# Autodesk Inventor assembly: hopper_assy
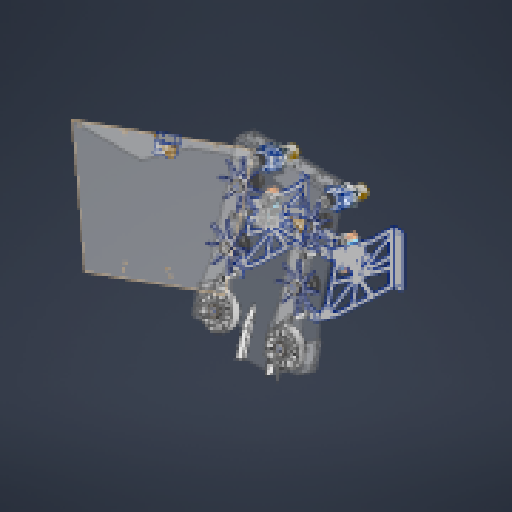
[picture p0: Inventor's stored thumbnail of the model, 512x512]
Saved by Autodesk Inventor 2024.3 (Build 283343000, 343)
## iProperties
Created: 2025-03-15
Part Number: hopper_assy
Document SubType Name: Assembly
Designer: Marcus Tannini
Author: Marcus Tannini
## Documents named in this file (31)
- C:\Users\jings\OneDrive\Desktop\FRC 5885\2025-Poseidon-Mechanical\hopper_assy.iam
- C:\Users\jings\OneDrive\Desktop\FRC 5885\2025-Poseidon-Mechanical\hopper_side_l.ipt
- C:\Users\jings\OneDrive\Desktop\FRC 5885\2025-Poseidon-Mechanical\hopper_side_r.ipt
- C:\Users\jings\OneDrive\Desktop\FRC 5885\2025-Poseidon-Mechanical\feeder_bottom_plate.ipt
- C:\Users\jings\OneDrive\Desktop\FRC 5885\2025-Poseidon-Mechanical\hopper_back.ipt
- C:\Users\jings\OneDrive\Desktop\FRC 5885\2025-Poseidon-Mechanical\hopper_side_bracket.ipt
- C:\Users\jings\OneDrive\Desktop\FRC 5885\2025-Poseidon-Mechanical\feeder_guide_plate.ipt
- C:\Users\jings\OneDrive\Desktop\FRC 5885\2025-Poseidon-Mechanical\am-5123 5IN 500IN Hex Bore Compliant Star.iam
- C:\Users\jings\OneDrive\Desktop\FRC 5885\2025-Poseidon-Mechanical\feeder_guide_plate_MIR.ipt
- C:\Users\jings\OneDrive\Desktop\FRC 5885\2025-Poseidon-Mechanical\CONTROLS,MOTOR,NEO,550.ipt
- C:\Users\jings\OneDrive\Desktop\FRC 5885\2025-Poseidon-Mechanical\VersaPlanetary v2 Dual Stage 10_1 with RS 550 (1).iam
- C:\Users\jings\OneDrive\Desktop\FRC 5885\2025-Poseidon-Mechanical\coral_guide.ipt
- C:\Users\jings\OneDrive\Desktop\FRC 5885\2025-Poseidon-Mechanical\coral_guide_MIR.ipt
- C:\Users\jings\OneDrive\Desktop\FRC 5885\2025-Poseidon-Mechanical\feeder_side_support_r.ipt
- C:\Users\jings\OneDrive\Desktop\FRC 5885\2025-Poseidon-Mechanical\feeder_side_support_l.ipt
- C:\Users\jings\OneDrive\Desktop\FRC 5885\2025-Poseidon-Mechanical\feeder_middle_brace.ipt
- C:\Users\jings\OneDrive\Desktop\FRC 5885\2025-Poseidon-Mechanical\2_1-2_hex_shaft.ipt
- C:\Users\jings\OneDrive\Desktop\FRC 5885\2025-Poseidon-Mechanical\PURCHASED,HEX_BEARING.ipt
- C:\Users\jings\OneDrive\Desktop\FRC 5885\2025-Poseidon-Mechanical\Bolt_Spacer.ipt
- C:\Users\jings\OneDrive\Desktop\FRC 5885\2025-Poseidon-Mechanical\CONTROLS,SPARK_MAX.ipt
- C:\Users\jings\OneDrive\Desktop\FRC 5885\2025-Poseidon-Mechanical\COVER,SPARKMAX.ipt
- C:\Users\jings\OneDrive\Desktop\FRC 5885\2025-Poseidon-Mechanical\16t 9mm.ipt
- C:\Users\jings\OneDrive\Desktop\FRC 5885\2025-Poseidon-Mechanical\19t 9mm.ipt
- C:\Users\jings\OneDrive\Desktop\FRC 5885\2025-Poseidon-Mechanical\29t 9mm.ipt
- C:\Users\jings\OneDrive\Desktop\FRC 5885\2025-Poseidon-Mechanical\am-3480 4IN 500Hex Bore Compliant Wheel REV2(1).iam
- C:\Users\jings\OneDrive\Desktop\FRC 5885\2025-Poseidon-Mechanical\1-2in_spacer.ipt
- C:\Users\jings\OneDrive\Desktop\FRC 5885\2025-Poseidon-Mechanical\hopper_fin.ipt
- C:\Users\jings\OneDrive\Desktop\FRC 5885\2025-Poseidon-Mechanical\hopper_fin_MIR.ipt
- C:\Users\jings\OneDrive\Desktop\FRC 5885\2025-Poseidon-Mechanical\1_CAD Library\CONTROLS,SPARK_MAX.ipt
- C:\Users\jings\OneDrive\Desktop\FRC 5885\2025-Poseidon-Mechanical\1_CAD Library\PURCHASED,GEARBOX,VERSA_PLANETARY,ADAPTER_CIM.ipt
- C:\Users\jings\OneDrive\Desktop\FRC 5885\2025-Poseidon-Mechanical\1_CAD Library\CONTROLS,MOTOR,NEO,V1.ipt
## Components (73 placed, 29 different names)
1. hopper_side_l:1
2. hopper_side_r:1
3. feeder_bottom_plate:1 — Mate:170, Mate:171, Mate:172, Mate:173, Mate:174, Mate:175
4. hopper_back:1
5. hopper_side_bracket:1
6. hopper_side_bracket:2
7. feeder_guide_plate:1
8. am-5123 5IN 500IN Hex Bore Compliant Star:1 [sub-assembly]
9. feeder_guide_plate_MIR:1
10. CONTROLS,MOTOR,NEO,550:1
11. VersaPlanetary v2 Dual Stage 10_1 with RS 550 (1):1 [sub-assembly]
12. coral_guide:1
13. coral_guide_MIR:1
14. feeder_side_support_r:1 — Mate:170, Mate:171, Mate:172
15. feeder_side_support_l:1 — Mate:173, Mate:174, Mate:175
16. feeder_middle_brace:1
17. 2_1-2_hex_shaft:1
18. PURCHASED,HEX_BEARING:1
19. 2_1-2_hex_shaft:2
20. PURCHASED,HEX_BEARING:2
21. am-5123 5IN 500IN Hex Bore Compliant Star:2 [sub-assembly]
22. 2_1-2_hex_shaft:3
23. PURCHASED,HEX_BEARING:3
24. am-5123 5IN 500IN Hex Bore Compliant Star:3 [sub-assembly]
25. 2_1-2_hex_shaft:4
26. PURCHASED,HEX_BEARING:4
27. am-5123 5IN 500IN Hex Bore Compliant Star:4 [sub-assembly]
28. CONTROLS,MOTOR,NEO,550:2
29. VersaPlanetary v2 Dual Stage 10_1 with RS 550 (1):2 [sub-assembly]
30. PURCHASED,HEX_BEARING:5
31. PURCHASED,HEX_BEARING:6
32. PURCHASED,HEX_BEARING:7
33. PURCHASED,HEX_BEARING:8
34. Bolt_Spacer:1
35. Bolt_Spacer:2
36. CONTROLS,SPARK_MAX:1
37. COVER,SPARKMAX:1
38. CONTROLS,SPARK_MAX:2
39. COVER,SPARKMAX:2
40. PURCHASED,HEX_BEARING:9
41. 2_1-2_hex_shaft:5
42. 2_1-2_hex_shaft:6
43. PURCHASED,HEX_BEARING:10
44. PURCHASED,HEX_BEARING:11
45. PURCHASED,HEX_BEARING:12
46. 16t 9mm:1
47. 16t 9mm:2
48. 16t 9mm:3
49. 16t 9mm:4
50. 19t 9mm:1
51. 19t 9mm:2
52. 19t 9mm:3
53. 19t 9mm:4
54. 29t 9mm:1
55. 29t 9mm:2
56. 29t 9mm:3
57. 29t 9mm:4
58. Bolt_Spacer:3
59. Bolt_Spacer:4
60. am-3480 4IN 500Hex Bore Compliant Wheel REV2(1):1 [sub-assembly]
61. am-3480 4IN 500Hex Bore Compliant Wheel REV2(1):2 [sub-assembly]
62. 1-2in_spacer:1
63. 1-2in_spacer:2
64. 1-2in_spacer:3
65. 1-2in_spacer:4
66. 1-2in_spacer:5
67. 1-2in_spacer:6
68. hopper_fin:1
69. hopper_fin_MIR:1
70. CONTROLS,SPARK_MAX:3
71. PURCHASED,GEARBOX,VERSA_PLANETARY,ADAPTER_CIM:1 — Insert:1, Insert:2, Insert:3, Insert:4
72. CONTROLS,MOTOR,NEO,V1:1 — Insert:1, Insert:2
73. VersaPlanetary v2 Dual Stage 10_1 with RS 550 (1):3 [sub-assembly] — Insert:3, Insert:4
## Relationships (197: Mate 168, Flush 20, RelateRotation 5, Insert 4)
- [Mate]: feeder_bottom_plate:1 ↔ hopper_back:1
- [Mate]: feeder_bottom_plate:1 ↔ hopper_back:1
- [Mate]: feeder_bottom_plate:1 ↔ hopper_back:1
- [Mate]: hopper_back:1 ↔ hopper_side_bracket:1
- [Mate]: hopper_back:1 ↔ hopper_side_bracket:1
- [Mate]: hopper_back:1 ↔ hopper_side_bracket:1
- [Mate]: hopper_side_l:1 ↔ hopper_side_bracket:1
- [Mate]: hopper_side_l:1 ↔ hopper_side_bracket:1
- [Mate]: hopper_side_l:1 ↔ hopper_side_bracket:1
- [Mate]: hopper_back:1 ↔ hopper_side_bracket:2
- [Mate]: hopper_back:1 ↔ hopper_side_bracket:2
- [Mate]: hopper_back:1 ↔ hopper_side_bracket:2
- [Mate]: hopper_side_r:1 ↔ hopper_side_bracket:2
- [Mate]: hopper_side_r:1 ↔ hopper_side_bracket:2
- [Mate]: hopper_side_r:1 ↔ hopper_side_bracket:2
- [Mate]: feeder_bottom_plate:1 ↔ feeder_guide_plate:1
- [Mate]: feeder_bottom_plate:1 ↔ feeder_guide_plate_MIR:1
- [Mate]: CONTROLS,MOTOR,NEO,550:1 ↔ VersaPlanetary v2 Dual Stage 10_1 with RS 550 (1):1
- [Mate]: CONTROLS,MOTOR,NEO,550:1 ↔ VersaPlanetary v2 Dual Stage 10_1 with RS 550 (1):1
- [Mate]: feeder_bottom_plate:1 ↔ VersaPlanetary v2 Dual Stage 10_1 with RS 550 (1):1
- [Flush]: feeder_bottom_plate:1 ↔ coral_guide:1
- [Mate]: feeder_bottom_plate:1 ↔ coral_guide:1
- [Flush]: feeder_bottom_plate:1 ↔ coral_guide_MIR:1
- [Mate]: feeder_bottom_plate:1 ↔ coral_guide_MIR:1
- [Mate] (69.85 mm): coral_guide:1 ↔ coral_guide_MIR:1
- [Flush] (11.1125 mm): feeder_bottom_plate:1 ↔ coral_guide:1
- [Mate]: feeder_side_support_r:1 ↔ feeder_middle_brace:1
- [Mate]: feeder_side_support_r:1 ↔ feeder_middle_brace:1
- [Mate]: feeder_side_support_r:1 ↔ feeder_middle_brace:1
- [Mate]: 2_1-2_hex_shaft:1 ↔ PURCHASED,HEX_BEARING:1
- [Mate]: 2_1-2_hex_shaft:1 ↔ PURCHASED,HEX_BEARING:1
- [Flush]: 2_1-2_hex_shaft:1 ↔ PURCHASED,HEX_BEARING:1
- [Mate]: 2_1-2_hex_shaft:2 ↔ PURCHASED,HEX_BEARING:2
- [Mate]: 2_1-2_hex_shaft:2 ↔ PURCHASED,HEX_BEARING:2
- [Flush]: 2_1-2_hex_shaft:2 ↔ PURCHASED,HEX_BEARING:2
- [Mate]: 2_1-2_hex_shaft:1 ↔ am-5123 5IN 500IN Hex Bore Compliant Star:2
- [Mate]: 2_1-2_hex_shaft:1 ↔ am-5123 5IN 500IN Hex Bore Compliant Star:2
- [Mate]: PURCHASED,HEX_BEARING:1 ↔ am-5123 5IN 500IN Hex Bore Compliant Star:2
- [Mate]: feeder_bottom_plate:1 ↔ feeder_guide_plate:1
- [Mate]: feeder_bottom_plate:1 ↔ feeder_guide_plate_MIR:1
- [Mate]: 2_1-2_hex_shaft:3 ↔ PURCHASED,HEX_BEARING:3
- [Mate]: 2_1-2_hex_shaft:3 ↔ PURCHASED,HEX_BEARING:3
- [Flush]: 2_1-2_hex_shaft:3 ↔ PURCHASED,HEX_BEARING:3
- [Mate]: 2_1-2_hex_shaft:3 ↔ am-5123 5IN 500IN Hex Bore Compliant Star:3
- [Mate]: 2_1-2_hex_shaft:3 ↔ am-5123 5IN 500IN Hex Bore Compliant Star:3
- [Mate]: PURCHASED,HEX_BEARING:3 ↔ am-5123 5IN 500IN Hex Bore Compliant Star:3
- [Mate]: 2_1-2_hex_shaft:4 ↔ PURCHASED,HEX_BEARING:4
- [Mate]: 2_1-2_hex_shaft:4 ↔ PURCHASED,HEX_BEARING:4
- [Flush]: 2_1-2_hex_shaft:4 ↔ PURCHASED,HEX_BEARING:4
- [Mate]: CONTROLS,MOTOR,NEO,550:2 ↔ VersaPlanetary v2 Dual Stage 10_1 with RS 550 (1):2
- [Mate]: CONTROLS,MOTOR,NEO,550:2 ↔ VersaPlanetary v2 Dual Stage 10_1 with RS 550 (1):2
- [Mate]: feeder_bottom_plate:1 ↔ VersaPlanetary v2 Dual Stage 10_1 with RS 550 (1):2
- [Mate]: feeder_bottom_plate:1 ↔ Bolt_Spacer:1
- [Mate]: feeder_bottom_plate:1 ↔ Bolt_Spacer:1
- [Mate]: feeder_bottom_plate:1 ↔ Bolt_Spacer:2
- [Mate]: feeder_bottom_plate:1 ↔ Bolt_Spacer:2
- [Mate]: CONTROLS,SPARK_MAX:1 ↔ COVER,SPARKMAX:1
- [Mate]: CONTROLS,SPARK_MAX:1 ↔ COVER,SPARKMAX:1
- [Mate]: CONTROLS,SPARK_MAX:1 ↔ COVER,SPARKMAX:1
- [Mate]: CONTROLS,SPARK_MAX:2 ↔ COVER,SPARKMAX:2
- [Mate]: CONTROLS,SPARK_MAX:2 ↔ COVER,SPARKMAX:2
- [Mate]: CONTROLS,SPARK_MAX:2 ↔ COVER,SPARKMAX:2
- [Mate]: feeder_side_support_r:1 ↔ COVER,SPARKMAX:1
- [Mate]: feeder_side_support_r:1 ↔ COVER,SPARKMAX:1
- [Mate]: feeder_side_support_r:1 ↔ CONTROLS,SPARK_MAX:1
- [Mate]: feeder_side_support_l:1 ↔ COVER,SPARKMAX:2
- [Mate]: feeder_side_support_l:1 ↔ COVER,SPARKMAX:2
- [Mate]: feeder_side_support_l:1 ↔ CONTROLS,SPARK_MAX:2
- [Mate]: feeder_bottom_plate:1 ↔ VersaPlanetary v2 Dual Stage 10_1 with RS 550 (1):1
- [Mate]: feeder_bottom_plate:1 ↔ VersaPlanetary v2 Dual Stage 10_1 with RS 550 (1):1
- [Mate]: feeder_bottom_plate:1 ↔ VersaPlanetary v2 Dual Stage 10_1 with RS 550 (1):2
- [Mate]: feeder_bottom_plate:1 ↔ VersaPlanetary v2 Dual Stage 10_1 with RS 550 (1):2
- [Mate]: PURCHASED,HEX_BEARING:9 ↔ 2_1-2_hex_shaft:6
- [Mate]: PURCHASED,HEX_BEARING:9 ↔ 2_1-2_hex_shaft:6
- [Flush]: PURCHASED,HEX_BEARING:9 ↔ 2_1-2_hex_shaft:6
- [Flush]: 2_1-2_hex_shaft:6 ↔ PURCHASED,HEX_BEARING:12
- [Mate]: 2_1-2_hex_shaft:6 ↔ PURCHASED,HEX_BEARING:12
- [Mate]: 2_1-2_hex_shaft:6 ↔ PURCHASED,HEX_BEARING:12
- [Flush]: 2_1-2_hex_shaft:5 ↔ PURCHASED,HEX_BEARING:10
- [Mate]: 2_1-2_hex_shaft:5 ↔ PURCHASED,HEX_BEARING:10
- [Mate]: 2_1-2_hex_shaft:5 ↔ PURCHASED,HEX_BEARING:10
- [Flush]: 2_1-2_hex_shaft:5 ↔ PURCHASED,HEX_BEARING:11
- [Mate]: 2_1-2_hex_shaft:5 ↔ PURCHASED,HEX_BEARING:11
- [Mate]: 2_1-2_hex_shaft:5 ↔ PURCHASED,HEX_BEARING:11
- [Mate]: feeder_guide_plate:1 ↔ PURCHASED,HEX_BEARING:10
- [Mate]: feeder_guide_plate:1 ↔ PURCHASED,HEX_BEARING:10
- [Mate]: feeder_bottom_plate:1 ↔ PURCHASED,HEX_BEARING:6
- [Mate]: feeder_bottom_plate:1 ↔ PURCHASED,HEX_BEARING:6
- [Mate]: feeder_bottom_plate:1 ↔ PURCHASED,HEX_BEARING:5
- [Mate]: feeder_bottom_plate:1 ↔ PURCHASED,HEX_BEARING:5
- [Mate]: feeder_guide_plate:1 ↔ PURCHASED,HEX_BEARING:2
- [Mate]: feeder_guide_plate:1 ↔ PURCHASED,HEX_BEARING:2
- [Mate]: feeder_guide_plate:1 ↔ PURCHASED,HEX_BEARING:1
- [Mate]: feeder_guide_plate:1 ↔ PURCHASED,HEX_BEARING:1
- [Flush]: am-5123 5IN 500IN Hex Bore Compliant Star:1 ↔ am-5123 5IN 500IN Hex Bore Compliant Star:2
- [Mate]: am-5123 5IN 500IN Hex Bore Compliant Star:1 ↔ 2_1-2_hex_shaft:5
- [Mate]: am-5123 5IN 500IN Hex Bore Compliant Star:1 ↔ 2_1-2_hex_shaft:5
- [Mate]: feeder_bottom_plate:1 ↔ PURCHASED,HEX_BEARING:8
- [Mate]: feeder_bottom_plate:1 ↔ PURCHASED,HEX_BEARING:8
- [Mate]: feeder_bottom_plate:1 ↔ PURCHASED,HEX_BEARING:7
- [Mate]: feeder_bottom_plate:1 ↔ PURCHASED,HEX_BEARING:7
- [Mate]: feeder_guide_plate_MIR:1 ↔ PURCHASED,HEX_BEARING:3
- [Mate]: feeder_guide_plate_MIR:1 ↔ PURCHASED,HEX_BEARING:3
- [Mate]: feeder_guide_plate_MIR:1 ↔ PURCHASED,HEX_BEARING:4
- [Mate]: feeder_guide_plate_MIR:1 ↔ PURCHASED,HEX_BEARING:4
- [Mate]: feeder_guide_plate_MIR:1 ↔ PURCHASED,HEX_BEARING:9
- [Mate]: feeder_guide_plate_MIR:1 ↔ PURCHASED,HEX_BEARING:9
- [Mate]: am-5123 5IN 500IN Hex Bore Compliant Star:4 ↔ 2_1-2_hex_shaft:6
- [Mate]: am-5123 5IN 500IN Hex Bore Compliant Star:4 ↔ 2_1-2_hex_shaft:6
- [Flush]: am-5123 5IN 500IN Hex Bore Compliant Star:1 ↔ am-5123 5IN 500IN Hex Bore Compliant Star:4
- [RelateRotation] (1 ul): 2_1-2_hex_shaft:3 ↔ 2_1-2_hex_shaft:6
- [RelateRotation] (1 ul): 2_1-2_hex_shaft:3 ↔ 2_1-2_hex_shaft:4
- [RelateRotation] (1 ul): 2_1-2_hex_shaft:5 ↔ 2_1-2_hex_shaft:6
- [RelateRotation] (1 ul): 2_1-2_hex_shaft:1 ↔ 2_1-2_hex_shaft:5
- [RelateRotation] (1 ul): 2_1-2_hex_shaft:1 ↔ 2_1-2_hex_shaft:2
- [Mate]: VersaPlanetary v2 Dual Stage 10_1 with RS 550 (1):1 ↔ 16t 9mm:2
- [Mate]: VersaPlanetary v2 Dual Stage 10_1 with RS 550 (1):1 ↔ 16t 9mm:2
- [Mate]: 2_1-2_hex_shaft:5 ↔ 16t 9mm:1
- [Mate]: 2_1-2_hex_shaft:5 ↔ 16t 9mm:1
- [Flush]: 16t 9mm:1 ↔ 16t 9mm:2
- [Mate]: VersaPlanetary v2 Dual Stage 10_1 with RS 550 (1):2 ↔ 16t 9mm:3
- [Mate]: VersaPlanetary v2 Dual Stage 10_1 with RS 550 (1):2 ↔ 16t 9mm:3
- [Flush]: 16t 9mm:2 ↔ 16t 9mm:3
- [Mate]: 2_1-2_hex_shaft:6 ↔ 16t 9mm:4
- [Mate]: 2_1-2_hex_shaft:6 ↔ 16t 9mm:4
- [Flush]: 16t 9mm:3 ↔ 16t 9mm:4
- [Mate]: 2_1-2_hex_shaft:6 ↔ 19t 9mm:3
- [Mate]: 16t 9mm:4 ↔ 19t 9mm:3
- [Mate]: 2_1-2_hex_shaft:6 ↔ 19t 9mm:3
- [Mate]: 2_1-2_hex_shaft:3 ↔ 19t 9mm:2
- [Flush]: 19t 9mm:2 ↔ 19t 9mm:3
- [Mate]: 2_1-2_hex_shaft:3 ↔ 19t 9mm:2
- [Mate]: 2_1-2_hex_shaft:5 ↔ 19t 9mm:1
- [Mate]: 16t 9mm:1 ↔ 19t 9mm:1
- [Mate]: 2_1-2_hex_shaft:5 ↔ 19t 9mm:1
- [Mate]: 2_1-2_hex_shaft:1 ↔ 19t 9mm:4
- [Flush]: 19t 9mm:1 ↔ 19t 9mm:4
- [Mate]: 2_1-2_hex_shaft:1 ↔ 19t 9mm:4
- [Mate]: 19t 9mm:4 ↔ 29t 9mm:2
- [Mate]: 2_1-2_hex_shaft:1 ↔ 29t 9mm:2
- [Mate]: 2_1-2_hex_shaft:1 ↔ 29t 9mm:2
- [Flush]: 29t 9mm:1 ↔ 29t 9mm:2
- [Mate]: 2_1-2_hex_shaft:2 ↔ 29t 9mm:1
- [Mate]: 2_1-2_hex_shaft:2 ↔ 29t 9mm:1
- [Mate]: 19t 9mm:2 ↔ 29t 9mm:3
- [Mate]: 2_1-2_hex_shaft:3 ↔ 29t 9mm:3
- [Mate]: 2_1-2_hex_shaft:3 ↔ 29t 9mm:3
- [Flush]: 29t 9mm:3 ↔ 29t 9mm:4
- [Mate]: 2_1-2_hex_shaft:4 ↔ 29t 9mm:4
- [Mate]: 2_1-2_hex_shaft:4 ↔ 29t 9mm:4
- [Mate]: PURCHASED,HEX_BEARING:12 ↔ 16t 9mm:4
- [Mate]: feeder_bottom_plate:1 ↔ Bolt_Spacer:3
- [Mate]: feeder_guide_plate:1 ↔ Bolt_Spacer:3
- [Mate]: feeder_bottom_plate:1 ↔ Bolt_Spacer:4
- [Mate]: feeder_guide_plate_MIR:1 ↔ Bolt_Spacer:4
- [Mate]: 2_1-2_hex_shaft:2 ↔ am-3480 4IN 500Hex Bore Compliant Wheel REV2(1):1
- [Mate]: 2_1-2_hex_shaft:2 ↔ am-3480 4IN 500Hex Bore Compliant Wheel REV2(1):1
- [Mate]: PURCHASED,HEX_BEARING:2 ↔ am-3480 4IN 500Hex Bore Compliant Wheel REV2(1):1
- [Mate]: 2_1-2_hex_shaft:4 ↔ am-3480 4IN 500Hex Bore Compliant Wheel REV2(1):2
- [Mate]: 2_1-2_hex_shaft:4 ↔ am-3480 4IN 500Hex Bore Compliant Wheel REV2(1):2
- [Mate]: PURCHASED,HEX_BEARING:4 ↔ am-3480 4IN 500Hex Bore Compliant Wheel REV2(1):2
- [Mate]: 2_1-2_hex_shaft:2 ↔ 1-2in_spacer:1
- [Mate]: 2_1-2_hex_shaft:2 ↔ 1-2in_spacer:1
- [Mate]: am-3480 4IN 500Hex Bore Compliant Wheel REV2(1):1 ↔ 1-2in_spacer:1
- [Mate]: 2_1-2_hex_shaft:1 ↔ 1-2in_spacer:2
- [Mate]: 2_1-2_hex_shaft:1 ↔ 1-2in_spacer:2
- [Mate]: 19t 9mm:4 ↔ 1-2in_spacer:2
- [Mate]: 2_1-2_hex_shaft:5 ↔ 1-2in_spacer:3
- [Mate]: 2_1-2_hex_shaft:5 ↔ 1-2in_spacer:3
- [Mate]: am-5123 5IN 500IN Hex Bore Compliant Star:1 ↔ 1-2in_spacer:3
- [Mate]: 2_1-2_hex_shaft:6 ↔ 1-2in_spacer:6
- [Mate]: 2_1-2_hex_shaft:6 ↔ 1-2in_spacer:6
- [Mate]: 19t 9mm:3 ↔ 1-2in_spacer:6
- [Mate]: 2_1-2_hex_shaft:3 ↔ 1-2in_spacer:5
- [Mate]: 2_1-2_hex_shaft:3 ↔ 1-2in_spacer:5
- [Mate]: 19t 9mm:2 ↔ 1-2in_spacer:5
- [Mate]: 2_1-2_hex_shaft:4 ↔ 1-2in_spacer:4
- [Mate]: 2_1-2_hex_shaft:4 ↔ 1-2in_spacer:4
- [Mate]: 29t 9mm:4 ↔ 1-2in_spacer:4
- [Mate]: feeder_bottom_plate:1 ↔ feeder_guide_plate_MIR:1
- [Mate]: feeder_bottom_plate:1 ↔ feeder_guide_plate:1
- [Mate]: hopper_back:1 ↔ hopper_fin:1
- [Mate]: hopper_back:1 ↔ hopper_fin:1
- [Mate]: hopper_back:1 ↔ hopper_fin_MIR:1
- [Mate]: hopper_back:1 ↔ hopper_fin_MIR:1
- [Mate]: hopper_back:1 ↔ hopper_fin_MIR:1
- [Mate]: hopper_back:1 ↔ hopper_fin:1
- Mate:170: feeder_bottom_plate:1 ↔ feeder_side_support_r:1
- Mate:171: feeder_bottom_plate:1 ↔ feeder_side_support_r:1
- Mate:172: feeder_bottom_plate:1 ↔ feeder_side_support_r:1
- Mate:173: feeder_bottom_plate:1 ↔ feeder_side_support_l:1
- Mate:174: feeder_bottom_plate:1 ↔ feeder_side_support_l:1
- Mate:175: feeder_bottom_plate:1 ↔ feeder_side_support_l:1
- Insert:1: PURCHASED,GEARBOX,VERSA_PLANETARY,ADAPTER_CIM:1 ↔ CONTROLS,MOTOR,NEO,V1:1
- Insert:2: PURCHASED,GEARBOX,VERSA_PLANETARY,ADAPTER_CIM:1 ↔ CONTROLS,MOTOR,NEO,V1:1
- Insert:3: PURCHASED,GEARBOX,VERSA_PLANETARY,ADAPTER_CIM:1 ↔ VersaPlanetary v2 Dual Stage 10_1 with RS 550 (1):3
- Insert:4: PURCHASED,GEARBOX,VERSA_PLANETARY,ADAPTER_CIM:1 ↔ VersaPlanetary v2 Dual Stage 10_1 with RS 550 (1):3
## Named parameters: d1224_d1196 = 0 mm, d1225_d1197 = 0 mm, d1226_d1198 = 0 mm, d1227_d1203 = 0 mm, d1228_d1204 = 0 mm, d1233_d1218 = 0 mm, d1237_d1199_d1196 = 0 mm, d1238_d1200_d1197 = 0 mm, d1239_d1201_d1198 = 0 mm, d1249_d1153_d967_d875_d873 = 0 mm, d1250_d1154_d968_d876_d874 = 0 mm, d1274_d169_d155 = 0 mm, d1275_d170_d156 = 0 mm, d1276_d171_d157 = 0 mm, d1277_d169_d155 = 0 mm, d1278_d170_d156 = 0 mm, d1279_d171_d157 = 0 mm, d1199_d1196 = 0 mm, d1200_d1197 = 0 mm, d1201_d1198 = 0 mm, d1153_d967_d875_d873 = 0 mm, d1154_d968_d876_d874 = 0 mm
